# Autodesk Inventor assembly: cap_cover
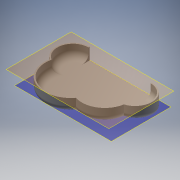
[picture p0: Inventor's stored thumbnail of the model, 180x180]
Saved by Autodesk Inventor 2018 (Build 220112000, 112)
## iProperties
Created: 2018-07-02
Part Number: cap_cover
Document SubType Name: Assembly
Designer: erwin
Author: erwin
## Documents named in this file (3)
- D:\GitHub\cloudberry-case\design\new\cap_cover.iam
- D:\GitHub\cloudberry-case\design\new\cap.ipt
- D:\GitHub\cloudberry-case\design\new\cap_cover.ipt
## Components (2 placed, 2 different names)
1. cap:1 — Flush:1, Flush:2, Flush:3
2. cap_cover:1 — Flush:1, Flush:2, Flush:3
## Relationships (3: Flush 3)
- Flush:1: cap:1 ↔ cap_cover:1
- Flush:2: cap:1 ↔ cap_cover:1
- Flush:3: cap:1 ↔ cap_cover:1
